# Autodesk Inventor assembly: Linear actuator v12_MIR_MIR1
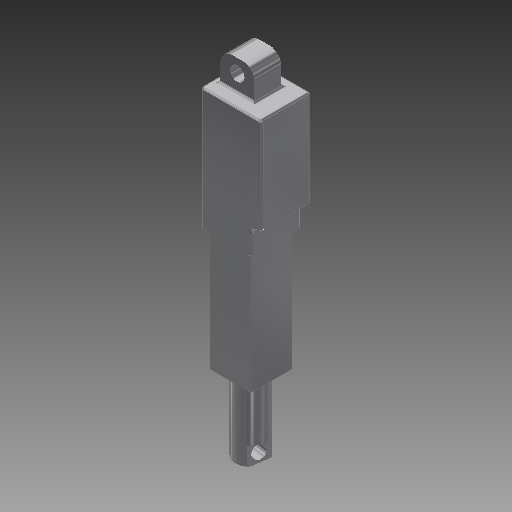
[picture p0: Inventor's stored thumbnail of the model, 512x512]
Saved by Autodesk Inventor 2019 (Build 230136000, 136)
## iProperties
Created: 2019-11-26
Part Number: Linear actuator v12_MIR_MIR1
Document SubType Name: Assembly
Designer: wojta
Title: Linear actuator v12 (3)
Author: Administrator
## Documents named in this file (3)
- C:\Users\wojta\Documents\Inventor\Reka\serwo\Linear actuator v12_MIR_MIR1.iam
- C:\Users\wojta\Documents\Inventor\Reka\serwo\Body serwo_MIR_MIR1.ipt
- C:\Users\wojta\Documents\Inventor\Reka\serwo\Push Rod_MIR_MIR1.ipt
## Components (2 placed, 2 different names)
1. Body serwo_MIR_MIR1:1 — Zestawiający:1
2. Push Rod_MIR_MIR1:1 — Zestawiający:1
## Relationships (1: Mate 1)
- Zestawiający:1 [Mate]: Body serwo_MIR_MIR1:1 ↔ Push Rod_MIR_MIR1:1
